# Autodesk Inventor assembly: 0 ASY PRS MAIN
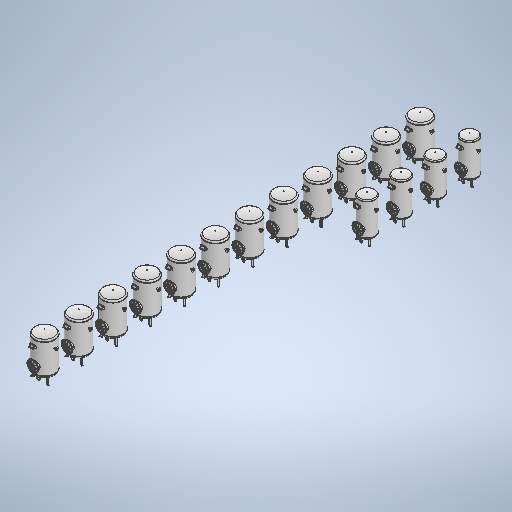
[picture p0: Inventor's stored thumbnail of the model, 512x512]
Saved by Autodesk Inventor 2026.2 (Build 302298000, 298)
## iProperties
Created: 2026-05-15
Part Number: 0 ASY PRS MAIN
Document SubType Name: Assembly
Designer: admin
Author: admin
## Documents named in this file (3)
- C:\Users\admin\Documents\Inventor\PRS-Purovsk\0 ASY PRS MAIN.iam
- C:\Users\admin\Documents\Inventor\PRS-Purovsk\ASY PRS 2 Filter column D1200.iam
- C:\Users\admin\Documents\Inventor\PRS-Purovsk\ASY PRS 2 Filter column D1200 940.iam
## Components (16 placed, 3 different names)
1. ASY PRS 2 Filter column D1200.iam:1 [sub-assembly] — Flush:2
2. ASY PRS 2 Filter column D1200:2 [sub-assembly]
3. ASY PRS 2 Filter column D1200:3 [sub-assembly]
4. ASY PRS 2 Filter column D1200:4 [sub-assembly]
5. ASY PRS 2 Filter column D1200:5 [sub-assembly]
6. ASY PRS 2 Filter column D1200:6 [sub-assembly]
7. ASY PRS 2 Filter column D1200:7 [sub-assembly]
8. ASY PRS 2 Filter column D1200:8 [sub-assembly]
9. ASY PRS 2 Filter column D1200:9 [sub-assembly]
10. ASY PRS 2 Filter column D1200:10 [sub-assembly]
11. ASY PRS 2 Filter column D1200:11 [sub-assembly]
12. ASY PRS 2 Filter column D1200:12 [sub-assembly]
13. ASY PRS 2 Filter column D1200 940:1 [sub-assembly]
14. ASY PRS 2 Filter column D1200 940:2 [sub-assembly]
15. ASY PRS 2 Filter column D1200 940:3 [sub-assembly]
16. ASY PRS 2 Filter column D1200 940:4 [sub-assembly]
## Component patterns: (12 elements, first: ASY PRS 2 Filter column D1200.iam:1), (4 elements, first: ASY PRS 2 Filter column D1200 940:1)
## Relationships (1: Flush 1)
- Flush:2: ASY PRS 2 Filter column D1200.iam:1
